# Autodesk Inventor assembly: basesinha
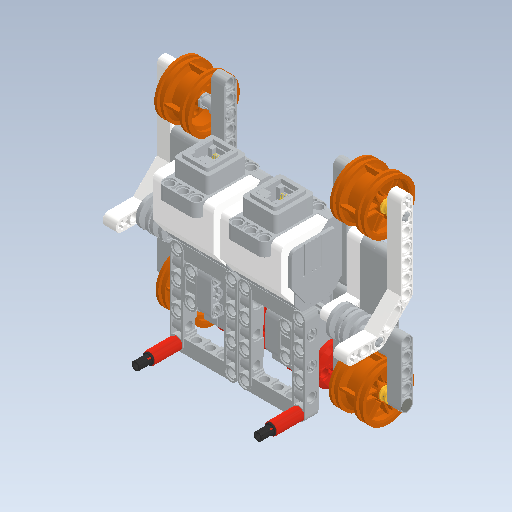
[picture p0: Inventor's stored thumbnail of the model, 512x512]
Saved by Autodesk Inventor 2020 (Build 240168000, 168)
## iProperties
Created: 2020-04-22
Part Number: basesinha
Document SubType Name: Assembly
Designer: gi-se
Author: gi-se
## Documents named in this file (33)
- C:\Users\gi-se\Desktop\rabo\3d\basesinha.iam
- C:\Users\gi-se\Desktop\rabo\3d\peças Lego\mindstorms\95658-EV3_Large_Motor v3.iam
- C:\Users\gi-se\Desktop\rabo\3d\peças Lego\conectores\Component2_6.ipt
- C:\Users\gi-se\Desktop\rabo\3d\peças Lego\vigas\Component2_3.ipt
- C:\Users\gi-se\Desktop\rabo\3d\peças Lego\vigas\Component2.ipt
- C:\Users\gi-se\Desktop\rabo\3d\peças Lego\conectores\Component2_5.ipt
- C:\Users\gi-se\Desktop\rabo\3d\peças Lego\eixos\Component1_8.ipt
- C:\Users\gi-se\Desktop\rabo\3d\peças Lego\vigas\Component2_32.ipt
- C:\Users\gi-se\Desktop\rabo\3d\peças Lego\vigas\Component2_18.ipt
- C:\Users\gi-se\Desktop\rabo\3d\peças Lego\conectores\Component2_13.ipt
- C:\Users\gi-se\Desktop\rabo\3d\peças Lego\conectores\Component2_7.ipt
- C:\Users\gi-se\Desktop\rabo\3d\peças Lego\rodas e egrenagens\56145_Wheel.ipt
- C:\Users\gi-se\Desktop\rabo\3d\peças Lego\eixos\Component1_7.ipt
- C:\Users\gi-se\Desktop\rabo\3d\peças Lego\vigas\Component2_6.ipt
- C:\Users\gi-se\Desktop\rabo\3d\peças Lego\vigas\Component2_7.ipt
- C:\Users\gi-se\Desktop\rabo\3d\peças Lego\rodas e egrenagens\13971-LtBluishGray.ipt
- C:\Users\gi-se\Desktop\rabo\3d\peças Lego\mindstorms\95658-EV3_Large_Motor v3_MIR.iam
- C:\Users\gi-se\Desktop\rabo\3d\peças Lego\conectores\Component2_6_MIR.ipt
- C:\Users\gi-se\Desktop\rabo\3d\peças Lego\vigas\Component2_3_MIR.ipt
- C:\Users\gi-se\Desktop\rabo\3d\peças Lego\vigas\Component2_MIR.ipt
- C:\Users\gi-se\Desktop\rabo\3d\peças Lego\conectores\Component2_5_MIR.ipt
- C:\Users\gi-se\Desktop\rabo\3d\peças Lego\eixos\Component1_8_MIR.ipt
- C:\Users\gi-se\Desktop\rabo\3d\peças Lego\vigas\Component2_32_MIR.ipt
- C:\Users\gi-se\Desktop\rabo\3d\peças Lego\vigas\Component2_18_MIR.ipt
- C:\Users\gi-se\Desktop\rabo\3d\peças Lego\conectores\Component2_7_MIR.ipt
- C:\Users\gi-se\Desktop\rabo\3d\peças Lego\rodas e egrenagens\56145_Wheel_MIR.ipt
- C:\Users\gi-se\Desktop\rabo\3d\peças Lego\conectores\Component2_13_MIR.ipt
- C:\Users\gi-se\Desktop\rabo\3d\peças Lego\eixos\Component1_7_MIR.ipt
- C:\Users\gi-se\Desktop\rabo\3d\peças Lego\vigas\Component2_6_MIR.ipt
- C:\Users\gi-se\Desktop\rabo\3d\peças Lego\vigas\Component2_7_MIR.ipt
- C:\Users\gi-se\Desktop\rabo\3d\peças Lego\rodas e egrenagens\13971-LtBluishGray_MIR.ipt
- C:\Users\gi-se\Desktop\rabo\3d\peças Lego\conectores\62462-Red.ipt
- C:\Users\gi-se\Desktop\rabo\3d\peças Lego\conectores\Component2.ipt
## Components (56 placed, 27 different names)
1. 95658-EV3_Large_Motor v3:1 [sub-assembly] — Coincidência:1, Coincidência:2, Coincidência:3, Coincidência:9, Coincidência:12, Coincidência:13, Coincidência:15, Alinhamento:2, Coincidência:21
2. Component2_6:2 — Coincidência:1, Coincidência:2, Coincidência:3, Coincidência:4, Coincidência:5, Coincidência:6, Coincidência:7, Coincidência:8
3. Component2_3:1 — Coincidência:4, Coincidência:5, Coincidência:6, Coincidência:7, Coincidência:8, Coincidência:110, Alinhamento:24
4. Component2:1 — Coincidência:11, Coincidência:12, Coincidência:14, Alinhamento:3, Alinhamento:4, Coincidência:46, Alinhamento:7, Coincidência:47
5. Component2_5:1 — Coincidência:9, Coincidência:11, Alinhamento:1, Coincidência:21
6. Component2_5:2 — Coincidência:13, Alinhamento:1, Coincidência:14, Coincidência:19, Coincidência:22, Alinhamento:5
7. Component1_8:1 — Coincidência:15, Alinhamento:2, Coincidência:16, Coincidência:31, Coincidência:35, Coincidência:37, Coincidência:51, Alinhamento:9
8. Component2_32:1 — Coincidência:16, Alinhamento:3, Alinhamento:4, Coincidência:18, Coincidência:25, Coincidência:29, Coincidência:30, Coincidência:32
9. Component2_18:2 — Coincidência:19, Coincidência:20, Coincidência:22, Alinhamento:5, Coincidência:27, Coincidência:28, Coincidência:53
10. Component2_5:3 — Coincidência:18, Coincidência:20, Coincidência:25, Coincidência:26
11. Component2_32:2 — Coincidência:23, Alinhamento:6, Coincidência:24, Coincidência:26, Coincidência:27, Alinhamento:10, Coincidência:52
12. Component2_32:3 — Coincidência:23, Alinhamento:6, Coincidência:24, Coincidência:28
13. Component2_5:4 — Coincidência:29, Coincidência:30
14. Component2_7:1 — Coincidência:31, Coincidência:32, Coincidência:50
15. 56145_Wheel:1 — Coincidência:35, Coincidência:38, Coincidência:50
16. Component2_13:2 — Coincidência:37, Coincidência:38
17. Component2_7:2 — Coincidência:44, Coincidência:47, Coincidência:49
18. 56145_Wheel:2 — Coincidência:42, Coincidência:49
19. Component2_13:4 — Coincidência:42, Coincidência:44, Coincidência:45
20. Component1_7:1 — Coincidência:45, Coincidência:46, Alinhamento:7, Coincidência:48, Alinhamento:8
21. Component1_7:2 — Alinhamento:11, Coincidência:53, Coincidência:56
22. Component2_6:3 — Coincidência:48, Alinhamento:8, Alinhamento:11, Coincidência:52, Coincidência:57
23. Component2_7:3 — Coincidência:51, Alinhamento:9, Alinhamento:10
24. 13971-LtBluishGray:1 — Coincidência:54, Coincidência:55, Coincidência:57
25. 13971-LtBluishGray:2 — Coincidência:54, Coincidência:55, Coincidência:56
26. 95658-EV3_Large_Motor v3_MIR:1 [sub-assembly] — Coincidência:58, Coincidência:59, Coincidência:60, Coincidência:66, Coincidência:67, Coincidência:69, Coincidência:71, Alinhamento:13, Coincidência:72
27. Component2_6_MIR:1 — Coincidência:58, Coincidência:59, Coincidência:60, Coincidência:61, Coincidência:62, Coincidência:63, Coincidência:64, Coincidência:65
28. Component2_3_MIR:1 — Coincidência:61, Coincidência:62, Coincidência:63, Coincidência:64, Coincidência:65, Coincidência:109, Alinhamento:23
29. Component2_MIR:1 — Coincidência:66, Coincidência:68, Coincidência:70, Alinhamento:14, Alinhamento:15, Coincidência:92, Alinhamento:18, Coincidência:97
30. Component2_5_MIR:1 — Coincidência:67, Coincidência:68, Coincidência:69, Alinhamento:12
31. Component2_5_MIR:2 — Coincidência:70, Alinhamento:12, Coincidência:71, Alinhamento:16, Coincidência:74, Coincidência:75
32. Component1_8_MIR:1 — Alinhamento:13, Coincidência:72, Coincidência:73, Coincidência:87, Coincidência:89, Coincidência:91, Alinhamento:22, Coincidência:102
33. Component2_32_MIR:1 — Alinhamento:14, Alinhamento:15, Coincidência:73, Coincidência:76, Coincidência:78, Coincidência:84, Coincidência:85, Coincidência:86
34. Component2_18_MIR:1 — Alinhamento:16, Coincidência:74, Coincidência:75, Coincidência:77, Coincidência:79, Coincidência:81, Coincidência:99
35. Component2_5_MIR:3 — Coincidência:76, Coincidência:77, Coincidência:78, Coincidência:80
36. Component2_32_MIR:2 — Coincidência:79, Coincidência:80, Coincidência:82, Alinhamento:17, Coincidência:83, Coincidência:100, Alinhamento:21
37. Component2_32_MIR:3 — Coincidência:81, Coincidência:82, Alinhamento:17, Coincidência:83
38. Component2_5_MIR:4 — Coincidência:84, Coincidência:85
39. Component2_7_MIR:1 — Coincidência:86, Coincidência:87, Coincidência:88
40. 56145_Wheel_MIR:1 — Coincidência:88, Coincidência:89, Coincidência:90
41. Component2_13_MIR:1 — Coincidência:90, Coincidência:91
42. Component2_7_MIR:2 — Coincidência:92, Coincidência:93, Coincidência:94
43. 56145_Wheel_MIR:2 — Coincidência:93, Coincidência:95, Coincidência:96
44. Component2_13_MIR:2 — Coincidência:94, Coincidência:95, Coincidência:96, Coincidência:98
45. Component1_7_MIR:1 — Alinhamento:18, Coincidência:97, Coincidência:98, Alinhamento:20, Coincidência:101
46. Component1_7_MIR:2 — Coincidência:99, Alinhamento:19, Coincidência:104
47. Component2_6_MIR:2 — Coincidência:100, Alinhamento:19, Alinhamento:20, Coincidência:101, Coincidência:103
48. Component2_7_MIR:3 — Alinhamento:21, Alinhamento:22, Coincidência:102
49. 13971-LtBluishGray_MIR:1 — Coincidência:103, Coincidência:105, Coincidência:106
50. 13971-LtBluishGray_MIR:2 — Coincidência:104, Coincidência:105, Coincidência:106
51. 62462-Red:1 — Coincidência:107, Coincidência:111, Coincidência:115, Coincidência:116
52. 62462-Red:2 — Coincidência:108, Coincidência:112, Coincidência:113, Coincidência:114
53. Component2:2 — Coincidência:108, Coincidência:109, Alinhamento:23, Coincidência:112
54. Component2:3 — Coincidência:107, Coincidência:110, Alinhamento:24, Coincidência:111
55. Component2:4 — Coincidência:113, Coincidência:114
56. Component2:5 — Coincidência:115, Coincidência:116
## Relationships (132: Mate 108, Flush 24)
- Coincidência:1 [Mate]: 95658-EV3_Large_Motor v3:1 ↔ Component2_6:2
- Coincidência:2 [Mate]: 95658-EV3_Large_Motor v3:1 ↔ Component2_6:2
- Coincidência:3 [Mate]: 95658-EV3_Large_Motor v3:1 ↔ Component2_6:2
- Coincidência:4 [Mate]: Component2_6:2 ↔ Component2_3:1
- Coincidência:5 [Mate]: Component2_6:2 ↔ Component2_3:1
- Coincidência:6 [Mate]: Component2_6:2 ↔ Component2_3:1
- Coincidência:7 [Mate]: Component2_6:2 ↔ Component2_3:1
- Coincidência:8 [Mate]: Component2_6:2 ↔ Component2_3:1
- Coincidência:9 [Mate]: 95658-EV3_Large_Motor v3:1 ↔ Component2_5:1
- Coincidência:11 [Mate]: Component2:1 ↔ Component2_5:1
- Coincidência:12 [Mate]: 95658-EV3_Large_Motor v3:1 ↔ Component2:1
- Coincidência:13 [Mate]: 95658-EV3_Large_Motor v3:1 ↔ Component2_5:2
- Alinhamento:1 [Flush]: Component2_5:1 ↔ Component2_5:2
- Coincidência:14 [Mate]: Component2:1 ↔ Component2_5:2
- Coincidência:15 [Mate]: 95658-EV3_Large_Motor v3:1 ↔ Component1_8:1
- Alinhamento:2 [Flush]: 95658-EV3_Large_Motor v3:1 ↔ Component1_8:1
- Coincidência:16 [Mate]: Component1_8:1 ↔ Component2_32:1
- Alinhamento:3 [Flush]: Component2:1 ↔ Component2_32:1
- Alinhamento:4 [Flush]: Component2:1 ↔ Component2_32:1
- Coincidência:18 [Mate]: Component2_32:1 ↔ Component2_5:3
- Coincidência:19 [Mate]: Component2_5:2 ↔ Component2_18:2
- Coincidência:20 [Mate]: Component2_18:2 ↔ Component2_5:3
- Coincidência:21 [Mate]: 95658-EV3_Large_Motor v3:1 ↔ Component2_5:1
- Coincidência:22 [Mate]: Component2_5:2 ↔ Component2_18:2
- Alinhamento:5 [Flush]: Component2_5:2 ↔ Component2_18:2
- Coincidência:23 [Mate]: Component2_32:2 ↔ Component2_32:3
- Alinhamento:6 [Flush]: Component2_32:2 ↔ Component2_32:3
- Coincidência:24 [Mate]: Component2_32:2 ↔ Component2_32:3
- Coincidência:25 [Mate]: Component2_32:1 ↔ Component2_5:3
- Coincidência:26 [Mate]: Component2_5:3 ↔ Component2_32:2
- Coincidência:27 [Mate]: Component2_18:2 ↔ Component2_32:2
- Coincidência:28 [Mate]: Component2_18:2 ↔ Component2_32:3
- Coincidência:29 [Mate]: Component2_32:1 ↔ Component2_5:4
- Coincidência:30 [Mate]: Component2_32:1 ↔ Component2_5:4
- Coincidência:31 [Mate]: Component1_8:1 ↔ Component2_7:1
- Coincidência:32 [Mate]: Component2_32:1 ↔ Component2_7:1
- Coincidência:35 [Mate]: Component1_8:1 ↔ 56145_Wheel:1
- Coincidência:37 [Mate]: Component1_8:1 ↔ Component2_13:2
- Coincidência:38 [Mate]: 56145_Wheel:1 ↔ Component2_13:2
- [Mate]: 56145_Wheel:2 ↔ Component2_13:4
- Coincidência:42 [Mate]: 56145_Wheel:2 ↔ Component2_13:4
- Coincidência:44 [Mate]: Component2_7:2 ↔ Component2_13:4
- Coincidência:45 [Mate]: Component2_13:4 ↔ Component1_7:1
- Coincidência:46 [Mate]: Component2:1 ↔ Component1_7:1
- Alinhamento:7 [Flush]: Component2:1 ↔ Component1_7:1
- Coincidência:47 [Mate]: Component2:1 ↔ Component2_7:2
- Coincidência:48 [Mate]: Component1_7:1 ↔ Component2_6:3
- Alinhamento:8 [Flush]: Component1_7:1 ↔ Component2_6:3
- Coincidência:49 [Mate]: Component2_7:2 ↔ 56145_Wheel:2
- Coincidência:50 [Mate]: Component2_7:1 ↔ 56145_Wheel:1
- Coincidência:51 [Mate]: Component1_8:1 ↔ Component2_7:3
- Alinhamento:9 [Flush]: Component1_8:1 ↔ Component2_7:3
- Alinhamento:10 [Flush]: Component2_32:2 ↔ Component2_7:3
- Alinhamento:11 [Flush]: Component1_7:2 ↔ Component2_6:3
- Coincidência:52 [Mate]: Component2_32:2 ↔ Component2_6:3
- Coincidência:53 [Mate]: Component2_18:2 ↔ Component1_7:2
- Coincidência:54 [Mate]: 13971-LtBluishGray:1 ↔ 13971-LtBluishGray:2
- Coincidência:55 [Mate]: 13971-LtBluishGray:1 ↔ 13971-LtBluishGray:2
- Coincidência:56 [Mate]: Component1_7:2 ↔ 13971-LtBluishGray:2
- Coincidência:57 [Mate]: Component2_6:3 ↔ 13971-LtBluishGray:1
- Coincidência:58 [Mate]: 95658-EV3_Large_Motor v3_MIR:1 ↔ Component2_6_MIR:1
- Coincidência:59 [Mate]: 95658-EV3_Large_Motor v3_MIR:1 ↔ Component2_6_MIR:1
- Coincidência:60 [Mate]: 95658-EV3_Large_Motor v3_MIR:1 ↔ Component2_6_MIR:1
- Coincidência:61 [Mate]: Component2_6_MIR:1 ↔ Component2_3_MIR:1
- Coincidência:62 [Mate]: Component2_6_MIR:1 ↔ Component2_3_MIR:1
- Coincidência:63 [Mate]: Component2_6_MIR:1 ↔ Component2_3_MIR:1
- Coincidência:64 [Mate]: Component2_6_MIR:1 ↔ Component2_3_MIR:1
- Coincidência:65 [Mate]: Component2_6_MIR:1 ↔ Component2_3_MIR:1
- Coincidência:66 [Mate]: 95658-EV3_Large_Motor v3_MIR:1 ↔ Component2_MIR:1
- Coincidência:67 [Mate]: 95658-EV3_Large_Motor v3_MIR:1 ↔ Component2_5_MIR:1
- Coincidência:68 [Mate]: Component2_MIR:1 ↔ Component2_5_MIR:1
- Coincidência:69 [Mate]: 95658-EV3_Large_Motor v3_MIR:1 ↔ Component2_5_MIR:1
- Coincidência:70 [Mate]: Component2_MIR:1 ↔ Component2_5_MIR:2
- Alinhamento:12 [Flush]: Component2_5_MIR:1 ↔ Component2_5_MIR:2
- Coincidência:71 [Mate]: 95658-EV3_Large_Motor v3_MIR:1 ↔ Component2_5_MIR:2
- Alinhamento:13 [Flush]: 95658-EV3_Large_Motor v3_MIR:1 ↔ Component1_8_MIR:1
- Coincidência:72 [Mate]: 95658-EV3_Large_Motor v3_MIR:1 ↔ Component1_8_MIR:1
- Alinhamento:14 [Flush]: Component2_MIR:1 ↔ Component2_32_MIR:1
- Alinhamento:15 [Flush]: Component2_MIR:1 ↔ Component2_32_MIR:1
- Coincidência:73 [Mate]: Component1_8_MIR:1 ↔ Component2_32_MIR:1
- Alinhamento:16 [Flush]: Component2_5_MIR:2 ↔ Component2_18_MIR:1
- Coincidência:74 [Mate]: Component2_5_MIR:2 ↔ Component2_18_MIR:1
- Coincidência:75 [Mate]: Component2_5_MIR:2 ↔ Component2_18_MIR:1
- Coincidência:76 [Mate]: Component2_32_MIR:1 ↔ Component2_5_MIR:3
- Coincidência:77 [Mate]: Component2_18_MIR:1 ↔ Component2_5_MIR:3
- Coincidência:78 [Mate]: Component2_32_MIR:1 ↔ Component2_5_MIR:3
- Coincidência:79 [Mate]: Component2_18_MIR:1 ↔ Component2_32_MIR:2
- Coincidência:80 [Mate]: Component2_5_MIR:3 ↔ Component2_32_MIR:2
- Coincidência:81 [Mate]: Component2_18_MIR:1 ↔ Component2_32_MIR:3
- Coincidência:82 [Mate]: Component2_32_MIR:2 ↔ Component2_32_MIR:3
- Alinhamento:17 [Flush]: Component2_32_MIR:2 ↔ Component2_32_MIR:3
- Coincidência:83 [Mate]: Component2_32_MIR:2 ↔ Component2_32_MIR:3
- Coincidência:84 [Mate]: Component2_32_MIR:1 ↔ Component2_5_MIR:4
- Coincidência:85 [Mate]: Component2_32_MIR:1 ↔ Component2_5_MIR:4
- Coincidência:86 [Mate]: Component2_32_MIR:1 ↔ Component2_7_MIR:1
- Coincidência:87 [Mate]: Component1_8_MIR:1 ↔ Component2_7_MIR:1
- Coincidência:88 [Mate]: Component2_7_MIR:1 ↔ 56145_Wheel_MIR:1
- Coincidência:89 [Mate]: Component1_8_MIR:1 ↔ 56145_Wheel_MIR:1
- Coincidência:90 [Mate]: 56145_Wheel_MIR:1 ↔ Component2_13_MIR:1
- Coincidência:91 [Mate]: Component1_8_MIR:1 ↔ Component2_13_MIR:1
- Coincidência:92 [Mate]: Component2_MIR:1 ↔ Component2_7_MIR:2
- Coincidência:93 [Mate]: Component2_7_MIR:2 ↔ 56145_Wheel_MIR:2
- Coincidência:94 [Mate]: Component2_7_MIR:2 ↔ Component2_13_MIR:2
- Coincidência:95 [Mate]: 56145_Wheel_MIR:2 ↔ Component2_13_MIR:2
- Coincidência:96 [Mate]: 56145_Wheel_MIR:2 ↔ Component2_13_MIR:2
- Alinhamento:18 [Flush]: Component2_MIR:1 ↔ Component1_7_MIR:1
- Coincidência:97 [Mate]: Component2_MIR:1 ↔ Component1_7_MIR:1
- Coincidência:98 [Mate]: Component2_13_MIR:2 ↔ Component1_7_MIR:1
- Coincidência:99 [Mate]: Component2_18_MIR:1 ↔ Component1_7_MIR:2
- Coincidência:100 [Mate]: Component2_32_MIR:2 ↔ Component2_6_MIR:2
- Alinhamento:19 [Flush]: Component1_7_MIR:2 ↔ Component2_6_MIR:2
- Alinhamento:20 [Flush]: Component1_7_MIR:1 ↔ Component2_6_MIR:2
- Coincidência:101 [Mate]: Component1_7_MIR:1 ↔ Component2_6_MIR:2
- Alinhamento:21 [Flush]: Component2_32_MIR:2 ↔ Component2_7_MIR:3
- Alinhamento:22 [Flush]: Component1_8_MIR:1 ↔ Component2_7_MIR:3
- Coincidência:102 [Mate]: Component1_8_MIR:1 ↔ Component2_7_MIR:3
- Coincidência:103 [Mate]: Component2_6_MIR:2 ↔ 13971-LtBluishGray_MIR:1
- Coincidência:104 [Mate]: Component1_7_MIR:2 ↔ 13971-LtBluishGray_MIR:2
- Coincidência:105 [Mate]: 13971-LtBluishGray_MIR:1 ↔ 13971-LtBluishGray_MIR:2
- Coincidência:106 [Mate]: 13971-LtBluishGray_MIR:1 ↔ 13971-LtBluishGray_MIR:2
- Coincidência:107 [Mate]: 62462-Red:1 ↔ Component2:3
- Coincidência:108 [Mate]: 62462-Red:2 ↔ Component2:2
- Coincidência:109 [Mate]: Component2_3_MIR:1 ↔ Component2:2
- Coincidência:110 [Mate]: Component2_3:1 ↔ Component2:3
- Alinhamento:23 [Flush]: Component2_3_MIR:1 ↔ Component2:2
- Alinhamento:24 [Flush]: Component2_3:1 ↔ Component2:3
- Coincidência:111 [Mate]: 62462-Red:1 ↔ Component2:3
- Coincidência:112 [Mate]: 62462-Red:2 ↔ Component2:2
- Coincidência:113 [Mate]: 62462-Red:2 ↔ Component2:4
- Coincidência:114 [Mate]: 62462-Red:2 ↔ Component2:4
- Coincidência:115 [Mate]: 62462-Red:1 ↔ Component2:5
- Coincidência:116 [Mate]: 62462-Red:1 ↔ Component2:5
## Named parameters: d47_d45 = 0 mm
